# Autodesk Inventor assembly: SHOT_1_002_ShooterAssembly
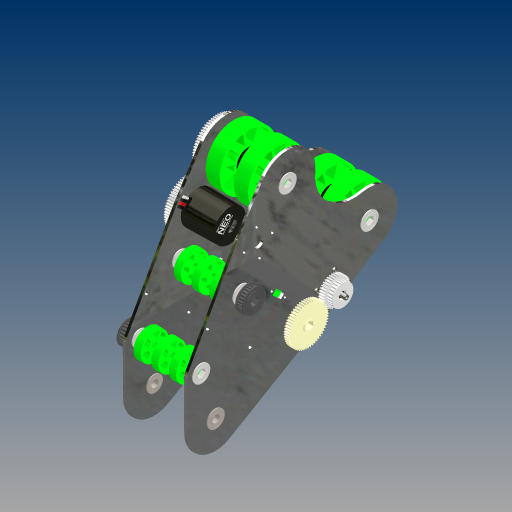
[picture p0: Inventor's stored thumbnail of the model, 512x512]
Saved by Autodesk Inventor 2024.3 (Build 283343000, 343)
## iProperties
Created: 2024-08-07
Part Number: SHOT_1_002_ShooterAssembly
Document SubType Name: Assembly
Designer: Kenji
Mass: 1474.99 g
Surface Area: 3908.93 cm^2
Volume: 710.058 cm^3
Density: 2.07728 g/cm^3
Author: Kenji
## Documents named in this file (15)
- C:\Users\Kenji\Documents\GitHub\1622-2024-Summer-CAD-A-Thon\Shooter\SHOT_1_002_ShooterAssembly.iam
- C:\Users\Kenji\Documents\GitHub\1622-2024-Summer-CAD-A-Thon\Shooter\SHOT_1_001_ShooterPlate.ipt
- C:\Users\Kenji\Documents\GitHub\1622-2024-Summer-CAD-A-Thon\COTS Library\Motion\Wheels\Compliant Wheels\4in compliant wheels\0.500in hex bore\COTS_am-3462_4indiameter_0.500inhexbore_durometer35A_CompliantWheel.ipt
- C:\Users\Kenji\Documents\GitHub\1622-2024-Summer-CAD-A-Thon\COTS Library\Motion\Bearings\COTS_WCP-0783_1.125ODHexBearing.ipt
- C:\Users\Kenji\Documents\GitHub\1622-2024-Summer-CAD-A-Thon\COTS Library\Motion\Bearings\COTS_WCP-0781_0.5ODCircularFlangedBearing.ipt
- C:\Users\Kenji\Documents\GitHub\1622-2024-Summer-CAD-A-Thon\COTS Library\Motors\COTS_REV-21-1650-V1.1_Neo1.1.ipt
- C:\Users\Kenji\Documents\GitHub\1622-2024-Summer-CAD-A-Thon\COTS Library\Motion\Wheels\Compliant Wheels\2in compliant wheels\0.500in hex bore\COTS_am-3462_2indiameter_0.500inhexbore_durometer35A_CompliantWheel.ipt
- C:\Users\Kenji\Documents\GitHub\1622-2024-Summer-CAD-A-Thon\COTS Library\Fasteners\Bolts\Button-Head\10-32\COTS_92949A265_1-2in long Stainless Steel Button Head Screw.ipt
- C:\Users\Kenji\Documents\GitHub\1622-2024-Summer-CAD-A-Thon\COTS Library\Motion\Pulleys\HTD5M\10mm Wide\COTS_HTD5M10mm24T_WCP-0564.ipt
- C:\Users\Kenji\Documents\GitHub\1622-2024-Summer-CAD-A-Thon\COTS Library\Structural Adapter\COTS_WCP-0794_0.5inshaftadapter.ipt
- C:\Users\Kenji\Documents\GitHub\1622-2024-Summer-CAD-A-Thon\COTS Library\Adapters\COTS_REV-21-1879_8mmKeyTo0.5Hex.ipt
- C:\Users\Kenji\Documents\GitHub\1622-2024-Summer-CAD-A-Thon\COTS Library\Motion\Gears\20DP gears\Aluminum\COTS_WCP-0171_66T.ipt
- C:\Users\Kenji\Documents\GitHub\1622-2024-Summer-CAD-A-Thon\Shooter\SHOT_1_004_66TGear-24TPulley.ipt
- C:\Users\Kenji\Documents\GitHub\1622-2024-Summer-CAD-A-Thon\COTS Library\Motion\Gears\20DP gears\Aluminum\COTS_WCP-0717_54T.ipt
- C:\Users\Kenji\Documents\GitHub\1622-2024-Summer-CAD-A-Thon\Shooter\SHOT_005_36TGear-24TPulley.ipt
## Components (47 placed, 14 different names)
1. SHOT_1_001_ShooterPlate:1 — Mate:140, Mate:141, Mate:142, Mate:143, Mate:144, Mate:148, Mate:150, Mate:151, Mate:152, Mate:153, Mate:155, Mate:160, Mate:161, Mate:163, Mate:164, Mate:165, Mate:166, Mate:167, Mate:168, Mate:169, Mate:170, Mate:171, Mate:172
2. SHOT_1_001_ShooterPlate:2 — Mate:140, Mate:141, Mate:145, Mate:147, Mate:149, Mate:156, Mate:157, Mate:158, Mate:159, Mate:173, Mate:174, Mate:175, Mate:176, Mate:177, Mate:178, Mate:179, Mate:180, Mate:181, Mate:183, Mate:192
3. COTS_WCP-0783_1.125ODHexBearing:1 — Mate:139, Flush:5, Mate:156, Mate:184
4. COTS_WCP-0783_1.125ODHexBearing:2 — Mate:146, Mate:147, Mate:149, Mate:193
5. COTS_WCP-0783_1.125ODHexBearing:3 — Mate:36, Mate:102, Flush:5
6. COTS_WCP-0783_1.125ODHexBearing:5 — Mate:50, Mate:136, Mate:155
7. COTS_WCP-0783_1.125ODHexBearing:9 — Mate:102, Flush:4, Mate:150, Mate:152, Mate:186, Mate:187
8. COTS_WCP-0783_1.125ODHexBearing:10 — Mate:31, Mate:104, Flush:4, Mate:151, Mate:188
9. COTS_WCP-0783_1.125ODHexBearing:11 — Mate:49, Mate:52, Mate:143, Mate:144, Mate:196, Mate:197
10. COTS_WCP-0783_1.125ODHexBearing:12 — Mate:154, Mate:157, Mate:189, Mate:190
11. COTS_WCP-0781_0.5ODCircularFlangedBearing:1 — Mate:138, Mate:158, Mate:159
12. COTS_WCP-0781_0.5ODCircularFlangedBearing:2 — Mate:138, Mate:160
13. COTS_REV-21-1650-V1.1_Neo1.1:1 — Mate:61, Mate:63, Mate:133, Mate:161, Mate:163, Mate:185
14. COTS_92949A265_1-2in long Stainless Steel Button Head Screw:1 — Mate:165, Mate:168, Mate:185
15. COTS_92949A265_1-2in long Stainless Steel Button Head Screw:2 — Mate:167, Mate:170
16. COTS_92949A265_1-2in long Stainless Steel Button Head Screw:3 — Mate:166, Mate:169
17. COTS_92949A265_1-2in long Stainless Steel Button Head Screw:4 — Mate:164, Mate:171
18. COTS_WCP-0794_0.5inshaftadapter:1 — Mate:61, Mate:63
19. COTS_WCP-0783_1.125ODHexBearing:13 — Mate:135, Mate:148, Mate:194, Mate:195
20. COTS_WCP-0783_1.125ODHexBearing:14 — Mate:134, Mate:145
21. COTS_REV-21-1650-V1.1_Neo1.1:2 — Mate:123, Mate:124, Mate:173, Mate:182, Mate:183, Mate:191
22. COTS_REV-21-1879_8mmKeyTo0.5Hex:1 — Mate:123, Mate:124
23. COTS_92949A265_1-2in long Stainless Steel Button Head Screw:5 — Mate:176, Mate:178, Mate:182
24. COTS_92949A265_1-2in long Stainless Steel Button Head Screw:6 — Mate:174, Mate:181
25. COTS_92949A265_1-2in long Stainless Steel Button Head Screw:7 — Mate:175, Mate:180
26. COTS_92949A265_1-2in long Stainless Steel Button Head Screw:8 — Mate:177, Mate:179
27. SHOT_1_004_66TGear-24TPulley:1 — Mate:133, Mate:172, Flush:6
28. COTS_WCP-0171_66T:1 — Mate:186, Mate:187
29. COTS_HTD5M10mm24T_WCP-0564:1 — Mate:188, Flush:6
30. COTS_WCP-0717_54T:1 — Mate:189, Mate:190
31. SHOT_005_36TGear-24TPulley:1 — Mate:191, Mate:192, Flush:7
32. COTS_HTD5M10mm24T_WCP-0564:2 — Mate:193, Flush:7
33. COTS_HTD5M10mm24T_WCP-0564:3 — Mate:194, Mate:195
34. COTS_HTD5M10mm24T_WCP-0564:4 — Mate:196, Mate:197
35. COTS_am-3462_4indiameter_0.500inhexbore_durometer35A_CompliantWheel:4 — Mate:36, Flush:3
36. COTS_am-3462_4indiameter_0.500inhexbore_durometer35A_CompliantWheel:1 — Mate:31, Flush:3, Mate:104
37. COTS_am-3462_4indiameter_0.500inhexbore_durometer35A_CompliantWheel:5
38. COTS_am-3462_4indiameter_0.500inhexbore_durometer35A_CompliantWheel:6 — Mate:139, Mate:184
39. COTS_am-3462_2indiameter_0.500inhexbore_durometer35A_CompliantWheel:2 — Mate:49, Flush:1, Mate:52
40. COTS_am-3462_2indiameter_0.500inhexbore_durometer35A_CompliantWheel:6 — Flush:2, Mate:135
41. COTS_am-3462_2indiameter_0.500inhexbore_durometer35A_CompliantWheel:1 — Mate:50, Flush:1, Flush:2, Mate:136
42. COTS_am-3462_2indiameter_0.500inhexbore_durometer35A_CompliantWheel:7 — Mate:142
43. COTS_am-3462_2indiameter_0.500inhexbore_durometer35A_CompliantWheel:8
44. COTS_am-3462_2indiameter_0.500inhexbore_durometer35A_CompliantWheel:9
45. COTS_am-3462_2indiameter_0.500inhexbore_durometer35A_CompliantWheel:10 — Mate:134
46. COTS_am-3462_2indiameter_0.500inhexbore_durometer35A_CompliantWheel:11 — Mate:146
47. COTS_am-3462_2indiameter_0.500inhexbore_durometer35A_CompliantWheel:12 — Mate:153, Mate:154
## Component patterns: (2 elements, first: COTS_am-3462_4indiameter_0.500inhexbore_durometer35A_CompliantWheel:4 + COTS_am-3462_4indiameter_0.500inhexbore_durometer35A_CompliantWheel:1), (3 elements, first: COTS_am-3462_2indiameter_0.500inhexbore_durometer35A_CompliantWheel:2 + COTS_am-3462_2indiameter_0.500inhexbore_durometer35A_CompliantWheel:6 + COTS_am-3462_2indiameter_0.500inhexbore_durometer35A_CompliantWheel:1)
## Relationships (81: Mate 74, Flush 7)
- Mate:31: COTS_WCP-0783_1.125ODHexBearing:10 ↔ COTS_am-3462_4indiameter_0.500inhexbore_durometer35A_CompliantWheel:1
- Mate:36: COTS_WCP-0783_1.125ODHexBearing:3 ↔ COTS_am-3462_4indiameter_0.500inhexbore_durometer35A_CompliantWheel:4
- Mate:49: COTS_WCP-0783_1.125ODHexBearing:11 ↔ COTS_am-3462_2indiameter_0.500inhexbore_durometer35A_CompliantWheel:2
- Mate:50: COTS_WCP-0783_1.125ODHexBearing:5 ↔ COTS_am-3462_2indiameter_0.500inhexbore_durometer35A_CompliantWheel:1
- Flush:1: COTS_am-3462_2indiameter_0.500inhexbore_durometer35A_CompliantWheel:2 ↔ COTS_am-3462_2indiameter_0.500inhexbore_durometer35A_CompliantWheel:1
- Flush:2: COTS_am-3462_2indiameter_0.500inhexbore_durometer35A_CompliantWheel:6 ↔ COTS_am-3462_2indiameter_0.500inhexbore_durometer35A_CompliantWheel:1
- Mate:52 (12.7 mm): COTS_WCP-0783_1.125ODHexBearing:11 ↔ COTS_am-3462_2indiameter_0.500inhexbore_durometer35A_CompliantWheel:2
- Mate:61: COTS_REV-21-1650-V1.1_Neo1.1:1 ↔ COTS_WCP-0794_0.5inshaftadapter:1
- Mate:63: COTS_REV-21-1650-V1.1_Neo1.1:1 ↔ COTS_WCP-0794_0.5inshaftadapter:1
- Mate:102: COTS_WCP-0783_1.125ODHexBearing:3 ↔ COTS_WCP-0783_1.125ODHexBearing:9
- Flush:3: COTS_am-3462_4indiameter_0.500inhexbore_durometer35A_CompliantWheel:4 ↔ COTS_am-3462_4indiameter_0.500inhexbore_durometer35A_CompliantWheel:1
- Mate:104 (12.7 mm): COTS_WCP-0783_1.125ODHexBearing:10 ↔ COTS_am-3462_4indiameter_0.500inhexbore_durometer35A_CompliantWheel:1
- Mate:123: COTS_REV-21-1650-V1.1_Neo1.1:2 ↔ COTS_REV-21-1879_8mmKeyTo0.5Hex:1
- Mate:124: COTS_REV-21-1650-V1.1_Neo1.1:2 ↔ COTS_REV-21-1879_8mmKeyTo0.5Hex:1
- Mate:133: COTS_REV-21-1650-V1.1_Neo1.1:1 ↔ SHOT_1_004_66TGear-24TPulley:1
- Mate:134: COTS_WCP-0783_1.125ODHexBearing:14 ↔ COTS_am-3462_2indiameter_0.500inhexbore_durometer35A_CompliantWheel:10
- Mate:135: COTS_WCP-0783_1.125ODHexBearing:13 ↔ COTS_am-3462_2indiameter_0.500inhexbore_durometer35A_CompliantWheel:6
- Mate:136: COTS_WCP-0783_1.125ODHexBearing:5 ↔ COTS_am-3462_2indiameter_0.500inhexbore_durometer35A_CompliantWheel:1
- Mate:138: COTS_WCP-0781_0.5ODCircularFlangedBearing:1 ↔ COTS_WCP-0781_0.5ODCircularFlangedBearing:2
- Mate:139: COTS_WCP-0783_1.125ODHexBearing:1 ↔ COTS_am-3462_4indiameter_0.500inhexbore_durometer35A_CompliantWheel:6
- Flush:4: COTS_WCP-0783_1.125ODHexBearing:9 ↔ COTS_WCP-0783_1.125ODHexBearing:10
- Flush:5: COTS_WCP-0783_1.125ODHexBearing:1 ↔ COTS_WCP-0783_1.125ODHexBearing:3
- Mate:140: SHOT_1_001_ShooterPlate:1 ↔ SHOT_1_001_ShooterPlate:2
- Mate:141: SHOT_1_001_ShooterPlate:1 ↔ SHOT_1_001_ShooterPlate:2
- Mate:142: SHOT_1_001_ShooterPlate:1 ↔ COTS_am-3462_2indiameter_0.500inhexbore_durometer35A_CompliantWheel:7
- Mate:143: SHOT_1_001_ShooterPlate:1 ↔ COTS_WCP-0783_1.125ODHexBearing:11
- Mate:144: SHOT_1_001_ShooterPlate:1 ↔ COTS_WCP-0783_1.125ODHexBearing:11
- Mate:145: SHOT_1_001_ShooterPlate:2 ↔ COTS_WCP-0783_1.125ODHexBearing:14
- Mate:146: COTS_WCP-0783_1.125ODHexBearing:2 ↔ COTS_am-3462_2indiameter_0.500inhexbore_durometer35A_CompliantWheel:11
- Mate:147: SHOT_1_001_ShooterPlate:2 ↔ COTS_WCP-0783_1.125ODHexBearing:2
- Mate:148: SHOT_1_001_ShooterPlate:1 ↔ COTS_WCP-0783_1.125ODHexBearing:13
- Mate:149: SHOT_1_001_ShooterPlate:2 ↔ COTS_WCP-0783_1.125ODHexBearing:2
- Mate:150: SHOT_1_001_ShooterPlate:1 ↔ COTS_WCP-0783_1.125ODHexBearing:9
- Mate:151: SHOT_1_001_ShooterPlate:1 ↔ COTS_WCP-0783_1.125ODHexBearing:10
- Mate:152: SHOT_1_001_ShooterPlate:1 ↔ COTS_WCP-0783_1.125ODHexBearing:9
- Mate:153: SHOT_1_001_ShooterPlate:1 ↔ COTS_am-3462_2indiameter_0.500inhexbore_durometer35A_CompliantWheel:12
- Mate:154: COTS_WCP-0783_1.125ODHexBearing:12 ↔ COTS_am-3462_2indiameter_0.500inhexbore_durometer35A_CompliantWheel:12
- Mate:155: SHOT_1_001_ShooterPlate:1 ↔ COTS_WCP-0783_1.125ODHexBearing:5
- Mate:156: SHOT_1_001_ShooterPlate:2 ↔ COTS_WCP-0783_1.125ODHexBearing:1
- Mate:157: SHOT_1_001_ShooterPlate:2 ↔ COTS_WCP-0783_1.125ODHexBearing:12
- Mate:158: SHOT_1_001_ShooterPlate:2 ↔ COTS_WCP-0781_0.5ODCircularFlangedBearing:1
- Mate:159: SHOT_1_001_ShooterPlate:2 ↔ COTS_WCP-0781_0.5ODCircularFlangedBearing:1
- Mate:160: SHOT_1_001_ShooterPlate:1 ↔ COTS_WCP-0781_0.5ODCircularFlangedBearing:2
- Mate:161: SHOT_1_001_ShooterPlate:1 ↔ COTS_REV-21-1650-V1.1_Neo1.1:1
- Mate:163: SHOT_1_001_ShooterPlate:1 ↔ COTS_REV-21-1650-V1.1_Neo1.1:1
- Mate:164: SHOT_1_001_ShooterPlate:1 ↔ COTS_92949A265_1-2in long Stainless Steel Button Head Screw:4
- Mate:165: SHOT_1_001_ShooterPlate:1 ↔ COTS_92949A265_1-2in long Stainless Steel Button Head Screw:1
- Mate:166: SHOT_1_001_ShooterPlate:1 ↔ COTS_92949A265_1-2in long Stainless Steel Button Head Screw:3
- Mate:167: SHOT_1_001_ShooterPlate:1 ↔ COTS_92949A265_1-2in long Stainless Steel Button Head Screw:2
- Mate:168: SHOT_1_001_ShooterPlate:1 ↔ COTS_92949A265_1-2in long Stainless Steel Button Head Screw:1
- Mate:169: SHOT_1_001_ShooterPlate:1 ↔ COTS_92949A265_1-2in long Stainless Steel Button Head Screw:3
- Mate:170: SHOT_1_001_ShooterPlate:1 ↔ COTS_92949A265_1-2in long Stainless Steel Button Head Screw:2
- Mate:171: SHOT_1_001_ShooterPlate:1 ↔ COTS_92949A265_1-2in long Stainless Steel Button Head Screw:4
- Mate:172: SHOT_1_001_ShooterPlate:1 ↔ SHOT_1_004_66TGear-24TPulley:1
- Mate:173: SHOT_1_001_ShooterPlate:2 ↔ COTS_REV-21-1650-V1.1_Neo1.1:2
- Mate:174: SHOT_1_001_ShooterPlate:2 ↔ COTS_92949A265_1-2in long Stainless Steel Button Head Screw:6
- Mate:175: SHOT_1_001_ShooterPlate:2 ↔ COTS_92949A265_1-2in long Stainless Steel Button Head Screw:7
- Mate:176: SHOT_1_001_ShooterPlate:2 ↔ COTS_92949A265_1-2in long Stainless Steel Button Head Screw:5
- Mate:177: SHOT_1_001_ShooterPlate:2 ↔ COTS_92949A265_1-2in long Stainless Steel Button Head Screw:8
- Mate:178: SHOT_1_001_ShooterPlate:2 ↔ COTS_92949A265_1-2in long Stainless Steel Button Head Screw:5
- Mate:179: SHOT_1_001_ShooterPlate:2 ↔ COTS_92949A265_1-2in long Stainless Steel Button Head Screw:8
- Mate:180: SHOT_1_001_ShooterPlate:2 ↔ COTS_92949A265_1-2in long Stainless Steel Button Head Screw:7
- Mate:181: SHOT_1_001_ShooterPlate:2 ↔ COTS_92949A265_1-2in long Stainless Steel Button Head Screw:6
- Mate:182: COTS_REV-21-1650-V1.1_Neo1.1:2 ↔ COTS_92949A265_1-2in long Stainless Steel Button Head Screw:5
- Mate:183: SHOT_1_001_ShooterPlate:2 ↔ COTS_REV-21-1650-V1.1_Neo1.1:2
- Mate:184 (12.7 mm): COTS_WCP-0783_1.125ODHexBearing:1 ↔ COTS_am-3462_4indiameter_0.500inhexbore_durometer35A_CompliantWheel:6
- Mate:185: COTS_REV-21-1650-V1.1_Neo1.1:1 ↔ COTS_92949A265_1-2in long Stainless Steel Button Head Screw:1
- Mate:186: COTS_WCP-0783_1.125ODHexBearing:9 ↔ COTS_WCP-0171_66T:1
- Mate:187: COTS_WCP-0783_1.125ODHexBearing:9 ↔ COTS_WCP-0171_66T:1
- Mate:188: COTS_WCP-0783_1.125ODHexBearing:10 ↔ COTS_HTD5M10mm24T_WCP-0564:1
- Flush:6: SHOT_1_004_66TGear-24TPulley:1 ↔ COTS_HTD5M10mm24T_WCP-0564:1
- Mate:189: COTS_WCP-0783_1.125ODHexBearing:12 ↔ COTS_WCP-0717_54T:1
- Mate:190: COTS_WCP-0783_1.125ODHexBearing:12 ↔ COTS_WCP-0717_54T:1
- Mate:191: COTS_REV-21-1650-V1.1_Neo1.1:2 ↔ SHOT_005_36TGear-24TPulley:1
- Mate:192: SHOT_1_001_ShooterPlate:2 ↔ SHOT_005_36TGear-24TPulley:1
- Mate:193: COTS_WCP-0783_1.125ODHexBearing:2 ↔ COTS_HTD5M10mm24T_WCP-0564:2
- Flush:7: SHOT_005_36TGear-24TPulley:1 ↔ COTS_HTD5M10mm24T_WCP-0564:2
- Mate:194: COTS_WCP-0783_1.125ODHexBearing:13 ↔ COTS_HTD5M10mm24T_WCP-0564:3
- Mate:195: COTS_WCP-0783_1.125ODHexBearing:13 ↔ COTS_HTD5M10mm24T_WCP-0564:3
- Mate:196: COTS_WCP-0783_1.125ODHexBearing:11 ↔ COTS_HTD5M10mm24T_WCP-0564:4
- Mate:197: COTS_WCP-0783_1.125ODHexBearing:11 ↔ COTS_HTD5M10mm24T_WCP-0564:4
